# Autodesk Inventor assembly: mascon-new
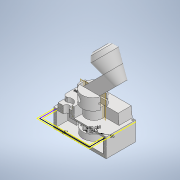
[picture p0: Inventor's stored thumbnail of the model, 180x180]
Saved by Autodesk Inventor 2021 (Build 250183000, 183)
## iProperties
Created: 2021-04-28
Part Number: mascon-new
Document SubType Name: Assembly
Designer: ben
Author: ben
## Documents named in this file (8)
- C:\Users\teh18\OneDrive\BVE Controller\r68-bve-mascon\mascon-new.iam
- C:\Users\teh18\OneDrive\BVE Controller\r68-bve-mascon\mascon.ipt
- C:\Users\teh18\OneDrive\BVE Controller\r68-bve-mascon\handle_base2.ipt
- C:\Users\teh18\OneDrive\BVE Controller\r68-bve-mascon\NotchPiston1.ipt
- C:\Users\teh18\OneDrive\BVE Controller\potentiometer-b10k-1.snapshot.2\PotentiometerB10K.ipt
- C:\Users\teh18\OneDrive\BVE Controller\r68-bve-mascon\PotHolder.ipt
- C:\Users\teh18\OneDrive\BVE Controller\r68-bve-mascon\handle-base\handle-base.iam
- C:\Users\teh18\OneDrive\BVE Controller\r68-bve-mascon\handle\handle.iam
## Components (7 placed, 7 different names)
1. mascon:1 — Flush:3, Mate:3, Mate:4, Tangent:1, Mate:8, Mate:9, handle turn
2. handle_base2:1 — Mate:10, Mate:11, Mate:12
3. NotchPiston1:1 — Flush:3
4. PotentiometerB10K:1 — Mate:4, Tangent:1
5. PotHolder:1 — Mate:3
6. handle-base:1 [sub-assembly] — Mate:8, Mate:9, handle pop, handle turn, Mate:10, Mate:11, Mate:12
7. handle:1 [sub-assembly] — handle pop
## Relationships (11: Mate 7, RevoluteJoint 2, Flush 1, Tangent 1)
- Flush:3: mascon:1 ↔ NotchPiston1:1
- Mate:3: mascon:1 ↔ PotHolder:1
- Mate:4: mascon:1 ↔ PotentiometerB10K:1
- Tangent:1: mascon:1 ↔ PotentiometerB10K:1
- Mate:8: mascon:1 ↔ handle-base:1
- Mate:9: mascon:1 ↔ handle-base:1
- handle pop [RevoluteJoint]: handle-base:1 ↔ handle:1
- handle turn [RevoluteJoint]: mascon:1 ↔ handle-base:1
- Mate:10: handle_base2:1 ↔ handle-base:1
- Mate:11: handle_base2:1 ↔ handle-base:1
- Mate:12: handle_base2:1 ↔ handle-base:1
